# Autodesk Inventor assembly: MTP16XL025-A-N12
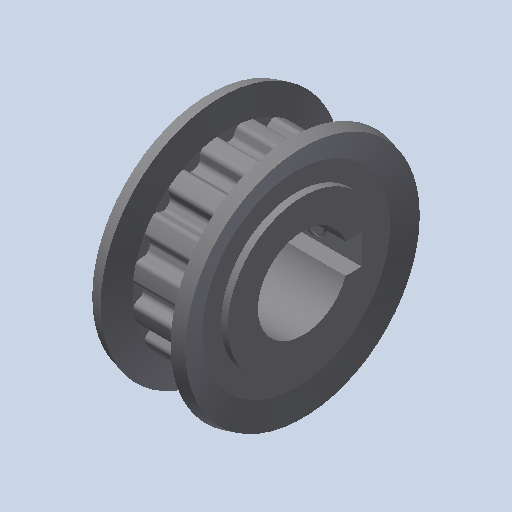
[picture p0: Inventor's stored thumbnail of the model, 512x512]
Saved by Autodesk Inventor 2025.1 (Build 291241000, 241)
## iProperties
Created: 2023-12-31
Part Number: MTP16XL025-A-N12
Catalog Web Link: www.cadenas.de
Description: ATP__XL025, ATP__XL031, ATP__ XL037, ATP__XL050, BTP__XL025, BTP__XL031, BTP__XL037, BTP__XL050, KTP__XL025, KTP__XL031, KTP__ XL037, KTP__XL050, NTP__XL025, NTP__XL031, NTP__ XL037, NTP__XL050, MTP__XL025, MTP__ XL037, MTP__XL050, MTPB__XL025, MTPB__ XL037, MTPB__XL050, MTPP__XL025, MTPP__ XL037, MTPP__XL050, STP__XL025, STP__XL031, STP__ XL037, STP__XL050, KATP__XL025, KATP__XL031, KATP__ XL037, KATP__XL050, KKTP__XL025, KKTP__XL031, KKTP__ XL037, KKTP__XL050-Timing Pulleys XL Type
Vendor: MISUMI
Document SubType Name: Assembly
Designer: psAdmin
Manufacturer: MISUMI
Mass: 5.03834 g
Surface Area: 39.109 cm^2
Volume: 5.03834 cm^3
Density: 1 g/cm^3
Category: PARTsolutions
Company: MISUMI
PSOL_IDENT_0: {$CADENAS_DATA/23d-libs/misumi/metric/51_timing_pulleys/mtp_xl_asmtab.prj},894 {VTYP=3D},{STYP=ASSTA
PSOL_IDENT_1: B},{NB=MTP16XL025-A-N12},{LINA=MTP16XL025-A-N12},{NN=ATP__XL025, ATP__XL031, ATP__ XL037, ATP__XL050
PSOL_IDENT_2: , BTP__XL025, BTP__XL031, BTP__XL037, BTP__XL050, KTP__XL025, KTP__XL031, KTP__ XL037, KTP__XL050, N
PSOL_IDENT_3: TP__XL025, NTP__XL031, NTP__ XL037, NTP__XL050, MTP__XL025, MTP__ XL037, MTP__XL050, MTPB__XL025, MT
PSOL_IDENT_4: PB__ XL037, MTPB__XL050, MTPP__XL025, MTPP__ XL037, MTPP__XL050, STP__XL025, STP__XL031, STP__ XL037
PSOL_IDENT_5: , STP__XL050, KATP__XL025, KATP__XL031, KATP__ XL037, KATP__XL050, KKTP__XL025, KKTP__XL031, KKTP__
PSOL_IDENT_6: XL037, KKTP__XL050},{DATE=06.01.2023 09:05:48},{GEOMDATE=06.01.2023 09:05:40},{VERSION=},{LINEID=30}
PSOL_IDENT_7: ,{WBVAR=MATP,ST,TNW,PS,SBS,DD,Z,J,Q,R,S,T,ALT1,ALT2,M,QSC,QFC,QTC,ALT3,K,KSC,KFC,KTC,ALT4,ZM,ZSC,ZFC
PSOL_IDENT_8: ,ZTC,ALT5,ALT6,ALT7,FC,ALT8,SRG,ALT9,BTC,TL,ALT10,TPC,ALT11,BC,ALT12,SLH,ALT13,BN},{WBNUMERIC=DD,Z,J
PSOL_IDENT_9: ,Q,R,S,T,QSC,QFC,QTC,K,KSC,KFC,KTC,ZSC,ZFC,ZTC,FC,SRG,BTC,TL,BC,SLH,BN}  {NB=MTP16XL025-A-N12},{LINA=
PSOL_IDENT_10: MTP16XL025-A-N12},{KT=DUMMY},{PN=MTP16XL025-A-N12},{TYPE=MTP},{MATP=S45C},{MATPALG= 'A2017','Aluminu
PSOL_IDENT_11: m Alloy 2000 series','S45C','1045 Carbon Steel Equivalent','SUS304','SUS304', 'A6000', '6000 Series
PSOL_IDENT_12: Aluminum Alloy' },{ST=-},{STALG= '-','-','BO','Black Oxide','ENP','Electroless Nickel Plating' },{NT=
PSOL_IDENT_13: 16},{TNW=XL025},{TNWALG= 'XL025','XL031','XL037','XL050' },{BW=6.4mm (1/4inch)},{PS=A},{PSALG= 'A','
PSOL_IDENT_14: B' },{SBS=N},{SBSALG= 'H','Round Hole','P','Round Hole + Tap','N','New JIS Keywayed Bore + Tap (Stan
PSOL_IDENT_15: dard)','NK','New JIS Keywayed Bore + Tap (width 4.0mm, height 1.8mm)','C','Old JIS Keywayed Bore + T
PSOL_IDENT_16: ap','V','Stepped Hole','Y','Both Ends Stepped Hole','WB','Double Stepped Hole' },{DD=12.00},{DDALG=[
PSOL_IDENT_17: 8:8/1],[10:13/1]},{DDHA=[5:6/1],6.35,[7:12/1],12.7,[13:16/1]},{DDPA=[5:6/1],6.35,[7:12/1],12.7,[13:1
PSOL_IDENT_18: 3/1]},{DDNA=[8:8/1],[10:13/1]},{DDNK=[10:10/1]},{DDCA=[10,12]},{DDVA=[5:6/1],6.35,[7:12/1],12.7,[13:
PSOL_IDENT_19: 14/1]},{DDY=[5:14/1]},{DDWB=[5:12/1]},{DDHB=},{DDPB=},{DDNB=},{DDCB=},{DDVFB=},{Z=0},{ZALG=[0]},{ZMI
PSOL_IDENT_20: N=14.000},{ZAMAX=16.000},{ZBMAX=0.000},{DDZ=12.000},{J=0.0},{JALG=[0]},{JMIN=2.000},{JMAX=10.500},{J
PSOL_IDENT_21: PN=},{Q=0},{QALG=[0]},{QRMIN=14.000},{QRMAX=16},{WBQMIN=16.000},{R=0},{RALG=[0]},{WBRMAX=-2.000},{S=
PSOL_IDENT_22: 0.0},{SALG=[0]},{SMAX=6.5},{T=0.0},{TALG=[0]},{TMAX=8},{SBSPN=-N12},{A=7.5},{W=12.5},{L=0},{PD=25.87
PSOL_IDENT_23: },{OD=25.36},{D=0},{DALG=17.000},{DE=20},{F=32},{E=20},{TT=1.6},{BBK=4.000},{TTK=1.8},{ALT1=},{ALT1A
PSOL_IDENT_24: LG= '','w/o KC90 (Set Screw Angle)','KC90','with KC90 (Set Screw Angle)' },{ANG=112.500},{ALT1PN=},{
PSOL_IDENT_25: ALT2=},{ALT2ALG= '','Not applicable' },{M=N/A},{MALG= 'N/A' },{MFTALG= 'N/A' },{MSALG= 'N/A' },{M3D=
PSOL_IDENT_26: 0.000},{KDML=0.000},{ML=0.000},{MUL=0.000},{PITCH=0.000},{QSC=0.0},{QSCALG=0},{QFC=0.0},{QFCALG=0},{
PSOL_IDENT_27: QTC=0.0},{QTCALG=0},{QPCDMIN=0.000},{QPCDMINALG=0.000},{QPCDMAX=16.000},{ALT2PN=},{TAP=0.000},{ALT3=
PSOL_IDENT_28: },{ALT3ALG= '','Not applicable' },{K=0.0},{KALG=0},{KMIN=4.000},{KFTMAX=0.000},{KSMAX=0.000},{KSC=0.
PSOL_IDENT_29: 0},{KSCALG=0},{KFC=0.0},{KFCALG=0},{KTC=0.0},{KTCALG=0},{KSCMIN=16.000},{KPCDMIN=16.000},{KPCDMAX=16
PSOL_IDENT_30: .000},{ALT3PN=},{ALT4=},{ALT4ALG= '','Not applicable' },{ALT4MIN=22.500},{ALT4MAX=9.500},{ZM=N/A},{Z
PSOL_IDENT_31: MALG= 'N/A' },{ZMFTALG= 'N/A' },{ZMSALG= 'N/A' },{ZMDD1=0.0},{ZMDD2=0.0},{ZMHH=0.0},{ZSC=0.0},{ZSCAL
PSOL_IDENT_32: G=[0]},{ZFC=0.0},{ZFCALG=[0]},{ZTC=0.0},{ZTCALG=[0]},{ZPCDMIN=0.000},{ZPCDMINALG=0.000},{ZPCDMAX=16.
PSOL_IDENT_33: 000},{ALT4PN=},{ALT5=},{ALT5ALG= '','w/o Flange not Attached','NFC','with NFC (Flange not Attached)'
PSOL_IDENT_34: },{ALT5PN=},{ALT6=},{ALT6ALG= '','w/o Flange Attached on One Side Only','RFC','with RFC (Flange Att
PSOL_IDENT_35: ached on The Boss Side Only)','LFC','with LFC (Flange Attached on The Opposite Side Only)' },{ALT6PN=
PSOL_IDENT_36: },{ALT7=},{ALT7ALG= '','w/o FC (Flange Cut)','FC','with FC (Flange Cut)' },{FC=0.0},{FCALG=0},{FCMIN=
PSOL_IDENT_37: 26.5},{FCMAX=30.0},{ALT7PN=},{ALT8=},{ALT8ALG= '','Not applicable' },{ALT8ALGALG=16.000},{ALT8DD2=0.
PSOL_IDENT_38: 000},{ALT8MM=0.000},{ALT8NN=0.000},{QC=0.000},{KC=0.000},{ZC=0.000},{SRG=0.0},{SRGALG=[0]},{SRGMAX=0
PSOL_IDENT_39: .000},{DD2=0.0},{MM=0.00},{NN=0.00},{ALT8PN=},{ALT9=},{ALT9ALG= '','Not applicable' },{BTC9=14.000},
PSOL_IDENT_40: {TL9=1.000},{BTC=0},{BTCALG=[0]},{TL=0.0},{TLALG=0},{TLMIN=1.000},{TLMAX=-13.000},{BTCL=0},{BTCD=0},
PSOL_IDENT_41: {ALT9PN=},{WLBCTL=12.500},{ALT10=},{ALT10ALG= '','w/o TPC (Tapped Hole Dimension)','TPC','with TPC (
PSOL_IDENT_42: Tapped Hole Dimension)' },{TPC=N/A},{TPCALG= 'N/A' },{TPCM=4.000},{ALT10PN=},{ALT11=},{ALT11ALG= '','
PSOL_IDENT_43: Not applicable' },{BC=0.0},{BCALG=0},{BCMIN=7},{BCMAX=-13},{M1WBC=6.25},{ALT11PN=},{KTT=4.88},{ALT12=
PSOL_IDENT_44: },{ALT12ALG= '','w/o SLH (Set Screw Length)','SLH','with SLH (Set Screw Length)' },{SLH=0},{SLHALG=[
PSOL_IDENT_45: 0]},{ALT12PN=},{ALT13=},{ALT13ALG= '', 'Not applicable' },{BN=0.0},{BNALG=0},{BNMIN=-12},{BNMAX=-2.5
PSOL_IDENT_46: },{ALT13PN=},{AC=M4x3},{M1=4.000},{M1L=3.000},{KEYA=1.000},{KEYB=0.000},{KEYM=1.000},{PPATH=mtp_xl/m
PSOL_IDENT_47: tp_xl_asmtpl.prj}
NB: MTP16XL025-A-N12
NN: 0
NT: 16
NBSYN: $PN.
LINA: MTP16XL025-A-N12
CATALOG: Misumi
PN: MTP16XL025-A-N12
MATP: 1045 Carbon Steel Equivalent
ST: -
TNW: XL025
BW: 6.4mm (1/4inch)
PS: A
SBS: New JIS Keywayed Bore + Tap (Standard)
DD: 12
Z: 0
J: 0
Q: 0
R: 0
S: 0
T: 0
A: 7.5
W: 12.5
L: 0
PD: 25.87
OD: 25.36
D: 0
F: 32
E: 20
TT: 1.6
ALT1: w/o KC90 (Set Screw Angle)
ALT2: Not applicable
M: N/A
QSC: 0
QFC: 0
QTC: 0
ALT3: Not applicable
K: 0
KSC: 0
KFC: 0
KTC: 0
ALT4: Not applicable
ZM: N/A
ZMDD1: 0
ZMDD2: 0
ZMHH: 0
ZSC: 0
ZFC: 0
ZTC: 0
ALT5: w/o Flange not Attached
ALT6: w/o Flange Attached on One Side Only
ALT7: w/o FC (Flange Cut)
FC: 0
ALT8: Not applicable
SRG: 0
DD2: 0
MM: 0
ALT9: Not applicable
BTC: 0
TL: 0
BTCL: 0
BTCD: 0
ALT10: w/o TPC (Tapped Hole Dimension)
TPC: N/A
ALT11: Not applicable
BC: 0
ALT12: w/o SLH (Set Screw Length)
SLH: 0
ALT13: Not applicable
BN: 0
AC: M4x3
SUPPLIER: MISUMI
ARTICLENO: MTP16XL025-A-N12
BOMINFO: MTP16XL025-A-N12
CREATOR: CADENAS GmbH
Title: MTP16XL025-A-N12
Author: Cadenas PARTsolutions
Comments: Timing Pulleys XL Type
## Documents named in this file (3)
- C:\Users\haruy\Documents\ロボコン\NHK2025\cad\nagahisa\dribl\R2-Rzvector\MTP16XL025-A-N12.iam
- C:\Users\haruy\Documents\ロボコン\NHK2025\cad\nagahisa\dribl\R2-Rzvector\MTP16XL025-A-N12_b.ipt
- C:\Users\haruy\Documents\ロボコン\NHK2025\cad\nagahisa\dribl\R2-Rzvector\SET-SCREW4-3.ipt
## Components (3 placed, 2 different names)
1. MTP16XL025-A-N12_b:1 — to_screw1_Z@1 <-> CP_Z@2, to_screw2_Z@1 <-> CP_Z@3
2. SET-SCREW4-3:1 — to_screw1_Z@1 <-> CP_Z@2
3. SET-SCREW4-3:2 — to_screw2_Z@1 <-> CP_Z@3
## Relationships (2: Mate 2)
- to_screw1_Z@1 <-> CP_Z@2 [Mate]: MTP16XL025-A-N12_b:1 ↔ SET-SCREW4-3:1
- to_screw2_Z@1 <-> CP_Z@3 [Mate]: MTP16XL025-A-N12_b:1 ↔ SET-SCREW4-3:2
